# Autodesk Inventor assembly: TreasureChestFinal-ver1-1111-2021
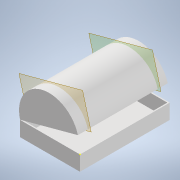
[picture p0: Inventor's stored thumbnail of the model, 180x180]
Saved by Autodesk Inventor 2021 (Build 250183000, 183)
## iProperties
Created: 2021-02-23
Part Number: TreasureChestFinal-ver1-1111-2021
Document SubType Name: Assembly
Designer: con_c_000
Author: con_c_000
## Documents named in this file (3)
- F:\PHRC CADD 2021\2021 Game Design Challenge\Treasure Chest\TreasureChestFinal-ver1-1111-2021.iam
- F:\PHRC CADD 2021\2021 Game Design Challenge\Treasure Chest\chestTop.ipt
- F:\PHRC CADD 2021\2021 Game Design Challenge\Treasure Chest\chestLower.ipt
## Components (2 placed, 2 different names)
1. chestTop:1 — Rotational:1
2. chestLower:1 — Rotational:1
## Relationships (1: RevoluteJoint 1)
- Rotational:1 [RevoluteJoint]: chestTop:1 ↔ chestLower:1
